# Autodesk Inventor assembly: Assembly KuggKroll
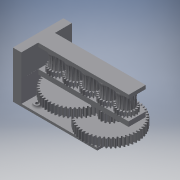
[picture p0: Inventor's stored thumbnail of the model, 180x180]
Saved by Autodesk Inventor 2016 (Build 200138000, 138)
## iProperties
Created: 2018-03-03
Part Number: Assembly KuggKroll
Document SubType Name: Assembly
Designer: Simon
Author: Simon
## Documents named in this file (10)
- D:\Cad\Gymnasieprojekt\Assembly KuggKroll.iam
- D:\Cad\Gymnasieprojekt\SUPERGEAR1.ipt
- D:\Cad\Gymnasieprojekt\SUPERGEAR2.ipt
- D:\Cad\Gymnasieprojekt\MotorKuggHolder.ipt
- D:\Cad\Gymnasieprojekt\SUPERGEAR12.ipt
- D:\Cad\Gymnasieprojekt\KruggHolder2.ipt
- D:\Cad\Gymnasieprojekt\Kroller Holder.ipt
- D:\Cad\Gymnasieprojekt\Kroller1.iam
- D:\Cad\Gymnasieprojekt\Kroller2.iam
- D:\Cad\Gymnasieprojekt\Kroller Holder2.ipt
## Components (13 placed, 9 different names)
1. SUPERGEAR1:1 — Insert:2, Insert:3, Insert:10, Insert:15
2. SUPERGEAR2:1 — Insert:4, Insert:5
3. SUPERGEAR2:2 — Insert:2, Insert:6, Insert:10
4. MotorKuggHolder:1 — Insert:3, Insert:4, Insert:8, Insert:15
5. SUPERGEAR12:1 — Insert:5
6. KruggHolder2:1 — Insert:6, Insert:13, Insert:14
7. Kroller Holder:1 — Insert:8, Insert:9, Insert:11, Insert:12, Insert:13, Insert:17, Insert:18
8. Kroller1:1 [sub-assembly] — Insert:9, Insert:14, Insert:16
9. Kroller2:1 [sub-assembly] — Insert:11
10. Kroller2:2 [sub-assembly] — Insert:12
11. Kroller Holder2:1 — Insert:16
12. Kroller2:3 [sub-assembly] — Insert:17
13. Kroller2:4 [sub-assembly] — Insert:18
## Relationships (16: Insert 16)
- Insert:2: SUPERGEAR1:1 ↔ SUPERGEAR2:2
- Insert:3: SUPERGEAR1:1 ↔ MotorKuggHolder:1
- Insert:4: SUPERGEAR2:1 ↔ MotorKuggHolder:1
- Insert:5: SUPERGEAR2:1 ↔ SUPERGEAR12:1
- Insert:6: SUPERGEAR2:2 ↔ KruggHolder2:1
- Insert:8: MotorKuggHolder:1 ↔ Kroller Holder:1
- Insert:9: Kroller Holder:1 ↔ Kroller1:1
- Insert:10: SUPERGEAR1:1 ↔ SUPERGEAR2:2
- Insert:11: Kroller Holder:1 ↔ Kroller2:1
- Insert:12: Kroller Holder:1 ↔ Kroller2:2
- Insert:13: KruggHolder2:1 ↔ Kroller Holder:1
- Insert:14: KruggHolder2:1 ↔ Kroller1:1
- Insert:15: SUPERGEAR1:1 ↔ MotorKuggHolder:1
- Insert:16: Kroller1:1 ↔ Kroller Holder2:1
- Insert:17: Kroller Holder:1 ↔ Kroller2:3
- Insert:18: Kroller Holder:1 ↔ Kroller2:4
